# Autodesk Inventor assembly: Chuck Assembly
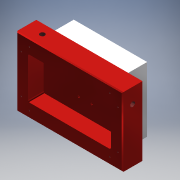
[picture p0: Inventor's stored thumbnail of the model, 180x180]
Saved by Autodesk Inventor 2019.4 (Build 234330000, 330)
## iProperties
Created: 2021-01-20
Part Number: Chuck Assembly
Document SubType Name: Assembly
Designer: caleb
Author: caleb
## Documents named in this file (3)
- C:\Users\cfang\Desktop\nebraska-silicon-lab\CAD\Wirebonder\Chuck Assembly.iam
- C:\Users\cfang\Desktop\nebraska-silicon-lab\CAD\Wirebonder\Chuck.ipt
- C:\Users\cfang\Desktop\nebraska-silicon-lab\CAD\Wirebonder\Chuck Spacer.ipt
## Components (2 placed, 2 different names)
1. Chuck:1 — Mate:1, Angle:1, Insert:1
2. Chuck Spacer:1 — Mate:1, Angle:1, Insert:1
## Relationships (3: Mate 1, Angle 1, Insert 1)
- Mate:1: Chuck:1 ↔ Chuck Spacer:1
- Angle:1 (0 deg): Chuck:1 ↔ Chuck Spacer:1
- Insert:1: Chuck:1 ↔ Chuck Spacer:1
